# Autodesk Inventor assembly: Skrzydlo sterowe
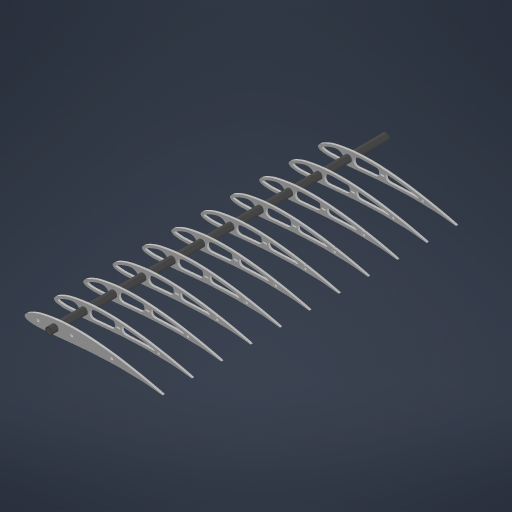
[picture p0: Inventor's stored thumbnail of the model, 512x512]
Saved by Autodesk Inventor 2023 (Build 270158000, 158)
## iProperties
Created: 2022-12-09
Part Number: Skrzydlo sterowe
Document SubType Name: Assembly
Designer: szykr
Author: szykr
## Documents named in this file (6)
- D:\Folder Instalacyjny\GitHub Pliki\Solaris\model\Skrzydlo sterowe.iam
- D:\Folder Instalacyjny\GitHub Pliki\Solaris\model\Wingspar trochemniejnizpol metrowy.ipt
- D:\Folder Instalacyjny\GitHub Pliki\Solaris\model\Żebro Montaż.ipt
- D:\Folder Instalacyjny\GitHub Pliki\Solaris\model\Żebro Default.ipt
- D:\Folder Instalacyjny\GitHub Pliki\Solaris\model\Zebro_lotka_serwo.iam
- D:\Folder Instalacyjny\GitHub Pliki\Solaris\model\Zebro_lotka_normal.iam
## Components (12 placed, 5 different names)
1. Wingspar trochemniejnizpol metrowy:1 — Insert:1
2. Żebro Montaż:1 — Insert:1, Angle:1, Insert:2, Insert:3, Insert:5
3. Zebro_lotka_serwo:1 [sub-assembly] — Insert:3, Insert:4
4. Żebro Default:1 — Insert:2
5. Żebro Default:2
6. Zebro_lotka_normal:1 [sub-assembly] — Insert:4
7. Zebro_lotka_normal:2 [sub-assembly]
8. Zebro_lotka_normal:3 [sub-assembly]
9. Zebro_lotka_normal:4 [sub-assembly]
10. Zebro_lotka_normal:5 [sub-assembly]
11. Żebro Default:3 — Insert:5
12. Żebro Default:4
## Component patterns: (2 elements, first: Żebro Default:1), (5 elements, first: Zebro_lotka_normal:1), (2 elements, first: Żebro Default:3)
## Relationships (6: Insert 5, Angle 1)
- Insert:1 (9 mm): Wingspar trochemniejnizpol metrowy:1 ↔ Żebro Montaż:1
- Angle:1 (270 deg): Żebro Montaż:1
- Insert:2 (42.4545 mm): Żebro Montaż:1 ↔ Żebro Default:1
- Insert:3 (127.3636 mm): Żebro Montaż:1 ↔ Zebro_lotka_serwo:1
- Insert:4 (42.4545 mm): Zebro_lotka_serwo:1 ↔ Zebro_lotka_normal:1
- Insert:5 (382.0909 mm): Żebro Montaż:1 ↔ Żebro Default:3
## Named parameters: ilosc_zeber_full = 11, ilosc_zeber_przed = 2, ilosc_lotek = 5, ilosc_zeber_po = 2, length_wingspara = 488 mm, length_true = 467 mm, spacing = 42.45455 mm
